# Autodesk Inventor assembly: activearm2
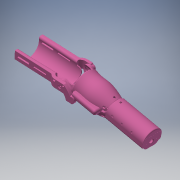
[picture p0: Inventor's stored thumbnail of the model, 180x180]
Saved by Autodesk Inventor 2016 (Build 200138000, 138)
## iProperties
Created: 2015-10-18
Part Number: activearm2
Document SubType Name: Assembly
Designer: master
Author: master
## Documents named in this file (7)
- C:\Users\master\Documents\!ActiveArm\activearm2.iam
- C:\Users\master\Documents\!ActiveArm\forearm.ipt
- C:\Users\master\Documents\!ActiveArm\L12.iam
- C:\Users\master\Documents\!ActiveArm\arm-cup.ipt
- C:\Users\master\Documents\!ActiveArm\ritarm\rit-triceps.ipt
- C:\Users\master\Documents\!ActiveArm\ritarm\hand-base.ipt
- C:\Users\master\Documents\!ActiveArm\armtop.ipt
## Components (6 placed, 6 different names)
1. forearm:1 — Cylindrical:1, Mate:1, Mate:2, Mate:3, Mate:6, Flush:1, Flush:2, Mate:8, Mate:9
2. L12:1 [sub-assembly] — Cylindrical:1, Mate:1, Mate:7
3. arm-cup:1 — Mate:2, Mate:3, Mate:4, Mate:5, Mate:6
4. rit-triceps:1 — Mate:4, Mate:5
5. hand-base:1 — Flush:1, Flush:2
6. armtop:1 — Mate:7, Mate:8, Mate:9
## Relationships (12: Mate 9, Flush 2, CylindricalJoint 1)
- Cylindrical:1: forearm:1 ↔ L12:1
- Mate:1: forearm:1 ↔ L12:1
- Mate:2: forearm:1 ↔ arm-cup:1
- Mate:3: forearm:1 ↔ arm-cup:1
- Mate:4: arm-cup:1 ↔ rit-triceps:1
- Mate:5: arm-cup:1 ↔ rit-triceps:1
- Mate:6: forearm:1 ↔ arm-cup:1
- Flush:1: forearm:1 ↔ hand-base:1
- Flush:2: forearm:1 ↔ hand-base:1
- Mate:7: L12:1 ↔ armtop:1
- Mate:8: forearm:1 ↔ armtop:1
- Mate:9: forearm:1 ↔ armtop:1
